# Autodesk Inventor assembly: Tamale Assembly Plate Assembly V3
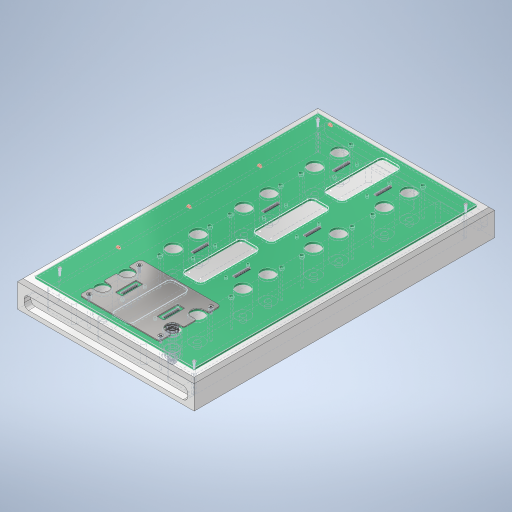
[picture p0: Inventor's stored thumbnail of the model, 512x512]
Saved by Autodesk Inventor 2023 (Build 270158000, 158)
## iProperties
Created: 2022-03-23
Part Number: Tamale Assembly Plate Assembly V3
Document SubType Name: Assembly
Designer: Caleb
Author: Caleb
## Documents named in this file (8)
- C:\Users\Caleb\Desktop\nebraska-silicon-lab\Hardware\ETL\Module Assembly\Tamale Assembly Plate V4\Tamale Assembly Plate Assembly V4.iam
- C:\Users\Caleb\Desktop\nebraska-silicon-lab\Hardware\ETL\Module Assembly\Tamale Assembly Plate V4\Tamale Assembly Plate V4.ipt
- C:\Users\Caleb\Desktop\nebraska-silicon-lab\Hardware\ETL\Module Assembly\Tamale Assembly Plate V4\spacer.ipt
- C:\Users\Caleb\Desktop\nebraska-silicon-lab\Hardware\ETL\Module Assembly\Tamale Assembly Plate V4\91771A054_Passivated 18-8 Stainless Steel Phillips Flat Head Screw.ipt
- C:\Users\Caleb\Desktop\nebraska-silicon-lab\Hardware\ETL\Module Assembly\Tamale Assembly Plate V4\90910A443_BUTTON HEAD TORX SCREWS.ipt
- C:\Users\Caleb\Desktop\nebraska-silicon-lab\Hardware\ETL\modules\throughput mockups\Throughput Mockup Assembly.iam
- C:\Users\Caleb\Desktop\nebraska-silicon-lab\Hardware\ETL\Module Assembly\Tamale Assembly Plate V4\5427A604_Vacuum Cup.ipt
- C:\Users\Caleb\Desktop\nebraska-silicon-lab\Hardware\ETL\Module Assembly\Tamale Assembly Plate V4\etl_assembly_plate_pcb_v4.ipt
## Components (13 placed, 7 different names)
1. Tamale Assembly Plate V4:1 — Insert:16
2. 90910A443_BUTTON HEAD TORX SCREWS:1
3. 90910A443_BUTTON HEAD TORX SCREWS:2
4. 90910A443_BUTTON HEAD TORX SCREWS:3
5. 90910A443_BUTTON HEAD TORX SCREWS:4
6. 91771A054_Passivated 18-8 Stainless Steel Phillips Flat Head Screw:3 — Insert:6
7. 91771A054_Passivated 18-8 Stainless Steel Phillips Flat Head Screw:1 — Insert:4
8. spacer:1 — Insert:4, Insert:5, Insert:6, Insert:7
9. 91771A054_Passivated 18-8 Stainless Steel Phillips Flat Head Screw:4 — Insert:7
10. 91771A054_Passivated 18-8 Stainless Steel Phillips Flat Head Screw:2 — Insert:5
11. etl_assembly_plate_pcb_v4:1
12. Throughput Mockup Assembly:1 [sub-assembly]
13. 5427A604_Vacuum Cup:1 — Insert:16
## Relationships (11: Insert 6, Flush 2, Mate 2, Angle 1)
- Insert:4: 91771A054_Passivated 18-8 Stainless Steel Phillips Flat Head Screw:1 ↔ spacer:1
- Insert:5: spacer:1 ↔ 91771A054_Passivated 18-8 Stainless Steel Phillips Flat Head Screw:2
- Insert:6: 91771A054_Passivated 18-8 Stainless Steel Phillips Flat Head Screw:3 ↔ spacer:1
- Insert:7: spacer:1 ↔ 91771A054_Passivated 18-8 Stainless Steel Phillips Flat Head Screw:4
- [Insert]: Tamale Assembly Plate V4:1 ↔ etl_assembly_plate_pcb_v4:1
- [Flush]: etl_assembly_plate_pcb_v4:1 ↔ Throughput Mockup Assembly:1
- [Flush]: etl_assembly_plate_pcb_v4:1 ↔ Throughput Mockup Assembly:1
- Insert:16: Tamale Assembly Plate V4:1 ↔ 5427A604_Vacuum Cup:1
- [Angle] (0 deg): Tamale Assembly Plate V4:1 ↔ etl_assembly_plate_pcb_v4:1
- [Mate] (0.7 mm): etl_assembly_plate_pcb_v4:1 ↔ Throughput Mockup Assembly:1
- [Mate]: spacer:1 ↔ etl_assembly_plate_pcb_v4:1
